# Autodesk Inventor assembly: test
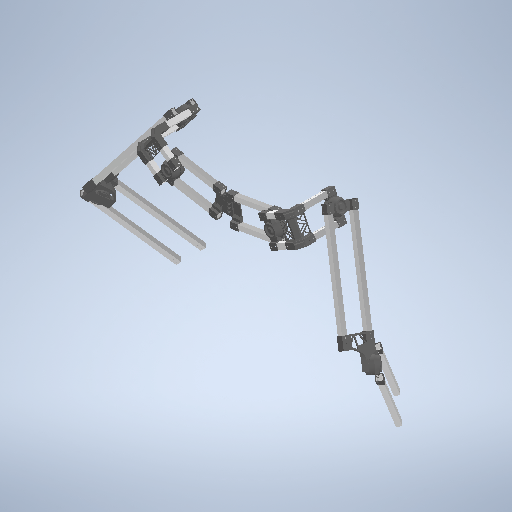
[picture p0: Inventor's stored thumbnail of the model, 512x512]
Saved by Autodesk Inventor 2026.1 (Build 301233020, 233B)
## iProperties
Created: 2026-02-01
Part Number: test
Document SubType Name: Assembly
Designer: hibik
Author: hibik
## Documents named in this file (15)
- C:\Users\hibik\Documents\Robomech\HR\controller\hard\body\Assy_body.iam
- C:\Users\hibik\Documents\Robomech\HR\controller\hard\body\back.ipt
- C:\Users\hibik\Documents\Robomech\HR\controller\hard\body\pole_setter.ipt
- C:\Users\hibik\Documents\Robomech\HR\controller\hard\body\body_size.ipt
- C:\Users\hibik\Documents\Robomech\HR\controller\hard\body\volume_upper.iam
- C:\Users\hibik\Documents\Robomech\HR\controller\hard\body\90_deg.ipt
- C:\Users\hibik\Documents\Robomech\HR\controller\hard\body\pipe_base2sholder_roll.ipt
- C:\Users\hibik\Documents\Robomech\HR\controller\hard\body\pipe_sholder_roll290deg.ipt
- C:\Users\hibik\Documents\Robomech\HR\controller\hard\body\pipe_sholder_90deg2pitch.ipt
- C:\Users\hibik\Documents\Robomech\HR\controller\hard\body\volume_under.iam
- C:\Users\hibik\Documents\Robomech\HR\controller\hard\body\pipe_sholder_pitch245deg.ipt
- C:\Users\hibik\Documents\Robomech\HR\controller\hard\body\45_deg_right.ipt
- C:\Users\hibik\Documents\Robomech\HR\controller\hard\body\volume_case_under.ipt
- C:\Users\hibik\Documents\Robomech\HR\controller\hard\body\pipe_elbow2hand.ipt
- C:\Users\hibik\Documents\Robomech\HR\controller\hard\body\45_deg_left.ipt
## Components (42 placed, 14 different names)
1. back:1 — フラッシュ:1, メイト:1, フラッシュ:2, メイト:2, フラッシュ:4, メイト:3, フラッシュ:6, メイト:4, フラッシュ:7, フラッシュ:8, フラッシュ:13, フラッシュ:14
2. pole_setter:1 — フラッシュ:1, メイト:1, フラッシュ:2, メイト:7, メイト:8, フラッシュ:9
3. pole_setter:2 — メイト:2, フラッシュ:4, 挿入:7, フラッシュ:13, 角度:6
4. pole_setter:3 — メイト:4, フラッシュ:7, フラッシュ:8, メイト:6, メイト:9, フラッシュ:10
5. pole_setter:4 — メイト:3, フラッシュ:6, フラッシュ:14, 挿入:8, 角度:7
6. body_size:1
7. volume_upper:1 [sub-assembly] — メイト:12, メイト:13, フラッシュ:12, 挿入:2, 角度:2, 挿入:10
8. 90_deg:1 — 角度:1, 挿入:3, 挿入:4, 挿入:5, 角度:3, 角度:4
9. pipe_base2sholder_roll:1 — メイト:7, メイト:8, フラッシュ:9, 挿入:9, 角度:8
10. pipe_base2sholder_roll:2 — メイト:6, メイト:9, フラッシュ:10
11. pipe_sholder_roll290deg:1 — メイト:12, メイト:13, フラッシュ:12, 角度:1, 挿入:3
12. pipe_sholder_roll290deg:2 — 挿入:2, 角度:2
13. volume_upper:3 [sub-assembly] — 挿入:12, 挿入:13, 挿入:14, 角度:10, 角度:11
14. pipe_sholder_90deg2pitch:1 — 挿入:4, 角度:3, 挿入:11, 角度:9
15. pipe_sholder_90deg2pitch:2 — 挿入:5, 角度:4
16. pipe_base2sholder_roll:3 — 挿入:7, 角度:6, 角度:20, 挿入:25
17. pipe_base2sholder_roll:4 — 挿入:8, 角度:7
18. volume_under:1 [sub-assembly] — 挿入:11, 角度:9, 挿入:12
19. volume_under:3 [sub-assembly] — 挿入:9, 角度:8, 挿入:10
20. pipe_sholder_pitch245deg:1 — 挿入:14, 角度:11
21. pipe_sholder_pitch245deg:2 — 挿入:13, 角度:10, 挿入:26, 角度:21
22. volume_upper:4 [sub-assembly]
23. 90_deg:2
24. pipe_sholder_roll290deg:3
25. pipe_sholder_roll290deg:4
26. volume_upper:5 [sub-assembly]
27. pipe_sholder_90deg2pitch:3
28. pipe_sholder_90deg2pitch:4
29. volume_under:4 [sub-assembly]
30. volume_under:5 [sub-assembly] — 角度:20, 挿入:25
31. pipe_sholder_pitch245deg:3 — 挿入:34, 角度:27
32. pipe_sholder_pitch245deg:4
33. 45_deg_right:1 — 挿入:26, 角度:21, 挿入:27, 角度:22
34. volume_case_under:1 — 挿入:27, 挿入:28, 角度:22
35. volume_upper:6 [sub-assembly] — 挿入:28, 挿入:29, 挿入:30, 角度:23, 角度:24
36. pipe_elbow2hand:1 — 挿入:29, 角度:23
37. pipe_elbow2hand:2 — 挿入:30, 角度:24
38. volume_case_under:2 — 挿入:35, 角度:28
39. volume_upper:7 [sub-assembly]
40. pipe_elbow2hand:3
41. pipe_elbow2hand:4
42. 45_deg_left:1 — 挿入:34, 角度:27, 挿入:35, 角度:28
## Relationships (82: Insert 32, Angle 26, Flush 12, Mate 12)
- フラッシュ:1 [Flush]: back:1 ↔ pole_setter:1
- メイト:1 [Mate]: back:1 ↔ pole_setter:1
- フラッシュ:2 [Flush]: back:1 ↔ pole_setter:1
- メイト:2 [Mate]: back:1 ↔ pole_setter:2
- フラッシュ:4 [Flush]: back:1 ↔ pole_setter:2
- メイト:3 [Mate]: back:1 ↔ pole_setter:4
- フラッシュ:6 [Flush]: back:1 ↔ pole_setter:4
- メイト:4 [Mate]: back:1 ↔ pole_setter:3
- フラッシュ:7 [Flush]: back:1 ↔ pole_setter:3
- フラッシュ:8 [Flush]: back:1 ↔ pole_setter:3
- メイト:6 [Mate]: pole_setter:3 ↔ pipe_base2sholder_roll:2
- メイト:7 [Mate]: pole_setter:1 ↔ pipe_base2sholder_roll:1
- メイト:8 [Mate]: pole_setter:1 ↔ pipe_base2sholder_roll:1
- フラッシュ:9 [Flush]: pole_setter:1 ↔ pipe_base2sholder_roll:1
- メイト:9 [Mate]: pole_setter:3 ↔ pipe_base2sholder_roll:2
- フラッシュ:10 [Flush]: pole_setter:3 ↔ pipe_base2sholder_roll:2
- メイト:12 [Mate]: volume_upper:1 ↔ pipe_sholder_roll290deg:1
- メイト:13 [Mate]: volume_upper:1 ↔ pipe_sholder_roll290deg:1
- フラッシュ:12 [Flush]: volume_upper:1 ↔ pipe_sholder_roll290deg:1
- 角度:1 [Angle] (0 deg): 90_deg:1 ↔ pipe_sholder_roll290deg:1
- 挿入:2 [Insert]: volume_upper:1 ↔ pipe_sholder_roll290deg:2
- 角度:2 [Angle] (0 deg): volume_upper:1 ↔ pipe_sholder_roll290deg:2
- 挿入:3 [Insert]: 90_deg:1 ↔ pipe_sholder_roll290deg:1
- 挿入:4 [Insert]: 90_deg:1 ↔ pipe_sholder_90deg2pitch:1
- 挿入:5 [Insert]: 90_deg:1 ↔ pipe_sholder_90deg2pitch:2
- 角度:3 [Angle] (0 deg): 90_deg:1 ↔ pipe_sholder_90deg2pitch:1
- 角度:4 [Angle] (0 deg): 90_deg:1 ↔ pipe_sholder_90deg2pitch:2
- 挿入:7 [Insert]: pole_setter:2 ↔ pipe_base2sholder_roll:3
- フラッシュ:13 [Flush]: back:1 ↔ pole_setter:2
- フラッシュ:14 [Flush]: back:1 ↔ pole_setter:4
- 挿入:8 [Insert]: pole_setter:4 ↔ pipe_base2sholder_roll:4
- 角度:6 [Angle] (0 deg): pole_setter:2 ↔ pipe_base2sholder_roll:3
- 角度:7 [Angle] (0 deg): pole_setter:4 ↔ pipe_base2sholder_roll:4
- 挿入:9 [Insert]: pipe_base2sholder_roll:1 ↔ volume_under:3
- 角度:8 [Angle] (0 deg): pipe_base2sholder_roll:1 ↔ volume_under:3
- 挿入:10 [Insert]: volume_upper:1 ↔ volume_under:3
- 挿入:11 [Insert]: pipe_sholder_90deg2pitch:1 ↔ volume_under:1
- 角度:9 [Angle] (0 deg): pipe_sholder_90deg2pitch:1 ↔ volume_under:1
- 挿入:12 [Insert]: volume_upper:3 ↔ volume_under:1
- 挿入:13 [Insert]: volume_upper:3 ↔ pipe_sholder_pitch245deg:2
- 挿入:14 [Insert]: volume_upper:3 ↔ pipe_sholder_pitch245deg:1
- 角度:10 [Angle] (0 deg): volume_upper:3 ↔ pipe_sholder_pitch245deg:2
- 角度:11 [Angle] (0 deg): volume_upper:3 ↔ pipe_sholder_pitch245deg:1
- [Mate]: volume_upper:4 ↔ pipe_sholder_roll290deg:3
- [Mate]: volume_upper:4 ↔ pipe_sholder_roll290deg:3
- [Flush]: volume_upper:4 ↔ pipe_sholder_roll290deg:3
- [Angle] (0 deg): 90_deg:2 ↔ pipe_sholder_roll290deg:3
- [Insert]: volume_upper:4 ↔ pipe_sholder_roll290deg:4
- [Angle] (0 deg): volume_upper:4 ↔ pipe_sholder_roll290deg:4
- [Insert]: 90_deg:2 ↔ pipe_sholder_roll290deg:3
- [Insert]: 90_deg:2 ↔ pipe_sholder_90deg2pitch:3
- [Insert]: 90_deg:2 ↔ pipe_sholder_90deg2pitch:4
- [Angle] (0 deg): 90_deg:2 ↔ pipe_sholder_90deg2pitch:3
- [Angle] (0 deg): 90_deg:2 ↔ pipe_sholder_90deg2pitch:4
- [Insert]: volume_upper:4 ↔ volume_under:5
- [Insert]: pipe_sholder_90deg2pitch:3 ↔ volume_under:4
- [Angle] (0 deg): pipe_sholder_90deg2pitch:3 ↔ volume_under:4
- [Insert]: volume_upper:5 ↔ volume_under:4
- [Insert]: volume_upper:5 ↔ pipe_sholder_pitch245deg:4
- [Insert]: volume_upper:5 ↔ pipe_sholder_pitch245deg:3
- [Angle] (0 deg): volume_upper:5 ↔ pipe_sholder_pitch245deg:4
- [Angle] (0 deg): volume_upper:5 ↔ pipe_sholder_pitch245deg:3
- 角度:20 [Angle] (0 deg): pipe_base2sholder_roll:3 ↔ volume_under:5
- 挿入:25 [Insert]: pipe_base2sholder_roll:3 ↔ volume_under:5
- 挿入:26 [Insert]: pipe_sholder_pitch245deg:2 ↔ 45_deg_right:1
- 角度:21 [Angle] (0 deg): pipe_sholder_pitch245deg:2 ↔ 45_deg_right:1
- 挿入:27 [Insert]: 45_deg_right:1 ↔ volume_case_under:1
- 挿入:28 [Insert]: volume_case_under:1 ↔ volume_upper:6
- 挿入:29 [Insert]: volume_upper:6 ↔ pipe_elbow2hand:1
- 挿入:30 [Insert]: volume_upper:6 ↔ pipe_elbow2hand:2
- 角度:22 [Angle] (0 deg): 45_deg_right:1 ↔ volume_case_under:1
- 角度:23 [Angle] (0 deg): volume_upper:6 ↔ pipe_elbow2hand:1
- 角度:24 [Angle] (0 deg): volume_upper:6 ↔ pipe_elbow2hand:2
- [Insert]: volume_case_under:2 ↔ volume_upper:7
- [Insert]: volume_upper:7 ↔ pipe_elbow2hand:3
- [Insert]: volume_upper:7 ↔ pipe_elbow2hand:4
- [Angle] (0 deg): volume_upper:7 ↔ pipe_elbow2hand:3
- [Angle] (0 deg): volume_upper:7 ↔ pipe_elbow2hand:4
- 挿入:34 [Insert]: pipe_sholder_pitch245deg:3 ↔ 45_deg_left:1
- 角度:27 [Angle] (0 deg): pipe_sholder_pitch245deg:3 ↔ 45_deg_left:1
- 挿入:35 [Insert]: volume_case_under:2 ↔ 45_deg_left:1
- 角度:28 [Angle] (0 deg): volume_case_under:2 ↔ 45_deg_left:1
## Named parameters: d71_d26 = 0 mm, d72_d27 = 0 mm, d73_d28 = 0 mm, d74_d30 = 0 deg, d75_d31 = 0 mm, d76_d32 = 0 deg, d77_d33 = 0 mm, d78_d42 = 0 mm, d79_d43 = 0 mm, d80_d44 = 0 deg, d81_d45 = 0 deg, d83_d67 = 0 mm, d84_d68 = 0 mm, d85_d69 = 0 deg, d86_d70 = 0 deg, d88_d63 = 0 mm, d89_d64 = 0 mm, d90_d65 = 0 deg, d91_d66 = 0 mm, d106_d100 = 0 mm, d107_d101 = 0 mm, d108_d102 = 0 mm, d109_d104 = 0 deg, d110_d105 = 0 deg
